# Autodesk Inventor assembly: 6 bar attachment_MIR
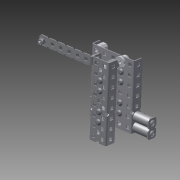
[picture p0: Inventor's stored thumbnail of the model, 180x180]
Saved by Autodesk Inventor 2014 SP1 (Build 180222100, 222)
## iProperties
Created: 2014-03-20
Part Number: 6 bar attachment_MIR
Document SubType Name: Assembly
Designer: Ryan
Author: Ryan
## Documents named in this file (16)
- C:\Users\Ryan\Desktop\sw\toss up 5th A bot\intake\6 bar attachment_MIR.iam
- C:\Users\Ryan\Desktop\sw\lib\Aperture VEX CAD Library\Metal\C Channel\5 x 7.ipt
- C:\Users\Ryan\Desktop\sw\lib\Aperture VEX CAD Library\Bearing Blocks\Bearing Block.ipt
- C:\Users\Ryan\Desktop\sw\lib\Aperture VEX CAD Library\Hardware\8-32\8-32_.500.ipt
- C:\Users\Ryan\Desktop\sw\lib\Aperture VEX CAD Library\Hardware\8-32\8-32 nylock.ipt
- C:\Users\Ryan\Desktop\sw\lib\Aperture VEX CAD Library\Metal\C Channel\2 x 8.ipt
- C:\Users\Ryan\Desktop\sw\lib\Aperture VEX CAD Library\Hardware\8-32\8-23_.750.ipt
- C:\Users\Ryan\Desktop\sw\lib\Aperture VEX CAD Library\Hardware\8-32\8-32 nylock_MIR14.ipt
- C:\Users\Ryan\Desktop\sw\lib\Aperture VEX CAD Library\Spacers\SPACER-0500-0375.ipt
- C:\Users\Ryan\Desktop\sw\lib\Aperture VEX CAD Library\Spacers\SPACER-0500-0250.ipt
- C:\Users\Ryan\Desktop\sw\lib\Aperture VEX CAD Library\Spacers\SPACER-0500-0125.ipt
- C:\Users\Ryan\Desktop\sw\lib\Aperture VEX CAD Library\Hardware\8-32\8-32_.375.ipt
- C:\Users\Ryan\Desktop\sw\lib\Aperture VEX CAD Library\Metal\Custom 1 bar\6 bend 1.ipt
- C:\Users\Ryan\Desktop\sw\lib\Aperture VEX CAD Library\Spacers\SPACER-0500-0500.ipt
- C:\Users\Ryan\Desktop\sw\lib\Aperture VEX CAD Library\Hardware\8-32\8-32_1.000.ipt
- C:\Users\Ryan\Desktop\sw\lib\Aperture VEX CAD Library\Metal\Custom 1 bar\1x2 bar.ipt
## Components (45 placed, 15 different names)
1. 5 x 7:1 — Mate:75, Mate:74, Mate:66, Mate:77, Mate:76, Mate:70, Mate:81, Mate:79, Mate:78, Mate:83, Flush:3, Flush:2, Mate:88, Mate:90, Mate:99, Mate:47, Mate:48, Mate:58, Mate:59, Mate:60, Mate:61, Flush:4
2. Bearing Block:1 — Mate:75, Mate:74, Mate:66, Mate:65, Mate:64, Mate:63, Mate:89
3. Bearing Block:2 — Mate:65, Mate:64, Mate:63, Mate:87, Mate:92, Mate:94, Mate:48
4. 2 x 8:1 — Flush:3, Flush:2, Mate:104, Mate:103, Mate:102, Flush:4, Mate:106
5. 8-23_.750:1 — Mate:88, Mate:87, Mate:91
6. 8-23_.750:2 — Mate:90, Mate:89, Mate:93
7. 8-32 nylock_MIR14:1 — Mate:92, Mate:91
8. 8-32 nylock:2 — Mate:94, Mate:93
9. SPACER-0500-0375:1 — Mate:96, Mate:95, Mate:101, Mate:49
10. SPACER-0500-0250:1 — Mate:96, Mate:95
11. SPACER-0500-0125:1 — Mate:101, Mate:100, Mate:99
12. 8-32_.375:1 — Mate:104, Mate:103, Mate:102, Mate:105, Mate:108, Mate:107
13. 8-32 nylock:3 — Mate:105, Mate:109
14. 6 bend 1:1 — Flush:4, Mate:109, Mate:108, Mate:107, Mate:106, Mate:112, Mate:111, Mate:110, Mate:114
15. 8-32_.375:2 — Mate:112, Mate:111, Mate:110, Mate:113
16. 8-32 nylock:4 — Mate:114, Mate:113
17. 1x2 bar:1 — Mate:56, Mate:57, Flush:4
18. Bearing Block:3 — Mate:77, Mate:76, Mate:70, Mate:82, Mate:85, Mate:100, Flush:3, Mate:47, Mate:49
19. Bearing Block:4 — Mate:81, Mate:79, Mate:78, Flush:3
20. Bearing Block:5
21. Bearing Block:6
22. 8-32_1.000:1 — Mate:56
23. SPACER-0500-0500:1 — Mate:57
24. SPACER-0500-0375:2 — Mate:59, Mate:60, Mate:61
25. 8-32 nylock:12 — Mate:58
26. 8-32_1.000:2
27. SPACER-0500-0500:2
28. SPACER-0500-0375:3
29. 8-32 nylock:13
30. 8-32_.500:1 — Mate:83, Mate:82, Mate:84
31. 8-32 nylock:1 — Mate:85, Mate:84
32. 8-32_.500:2
33. 8-32 nylock:5
34. 8-32_.500:3
35. 8-32 nylock:6
36. 8-32_.500:4
37. 8-32 nylock:7
38. 8-32_.500:5
39. 8-32 nylock:8
40. 8-32_.500:6
41. 8-32 nylock:9
42. 8-32_.500:7
43. 8-32 nylock:10
44. 8-32_.500:8
45. 8-32 nylock:11
## Component patterns: (2 elements, first: Bearing Block:3 + Bearing Block:4), (2 elements, first: 8-32_1.000:1 + SPACER-0500-0500:1 + SPACER-0500-0375:2 + 8-32 nylock:12), (4 elements, first: 8-32_.500:1 + 8-32 nylock:1), Component Pattern 1:2 (4 elements)
## Relationships (62: Mate 58, Flush 4)
- Mate:75 (2.3114 mm): 5 x 7:1 ↔ Bearing Block:1
- Mate:74 (2.3114 mm): 5 x 7:1 ↔ Bearing Block:1
- Mate:66: 5 x 7:1 ↔ Bearing Block:1
- Mate:65: Bearing Block:1 ↔ Bearing Block:2
- Mate:64: Bearing Block:1 ↔ Bearing Block:2
- Mate:63: Bearing Block:1 ↔ Bearing Block:2
- Mate:77 (2.3114 mm): 5 x 7:1 ↔ Bearing Block:3
- Mate:76 (2.3114 mm): 5 x 7:1 ↔ Bearing Block:3
- Mate:70: 5 x 7:1 ↔ Bearing Block:3
- Mate:81 (2.3114 mm): 5 x 7:1 ↔ Bearing Block:4
- Mate:79 (2.3114 mm): 5 x 7:1 ↔ Bearing Block:4
- Mate:78: 5 x 7:1 ↔ Bearing Block:4
- Mate:83: 5 x 7:1 ↔ 8-32_.500:1
- Mate:82: Bearing Block:3 ↔ 8-32_.500:1
- Mate:85: Bearing Block:3 ↔ 8-32 nylock:1
- Mate:84: 8-32_.500:1 ↔ 8-32 nylock:1
- Flush:3 [Mate]: 5 x 7:1 ↔ 2 x 8:1
- Flush:2: 5 x 7:1 ↔ 2 x 8:1
- Mate:88: 5 x 7:1 ↔ 8-23_.750:1
- Mate:87: Bearing Block:2 ↔ 8-23_.750:1
- Mate:90: 5 x 7:1 ↔ 8-23_.750:2
- Mate:89: Bearing Block:1 ↔ 8-23_.750:2
- Mate:92: Bearing Block:2 ↔ 8-32 nylock_MIR14:1
- Mate:91: 8-23_.750:1 ↔ 8-32 nylock_MIR14:1
- Mate:94: Bearing Block:2 ↔ 8-32 nylock:2
- Mate:93: 8-23_.750:2 ↔ 8-32 nylock:2
- Mate:96: SPACER-0500-0375:1 ↔ SPACER-0500-0250:1
- Mate:95: SPACER-0500-0375:1 ↔ SPACER-0500-0250:1
- Mate:101 (7.5184 mm): SPACER-0500-0375:1 ↔ SPACER-0500-0125:1
- Mate:100: SPACER-0500-0125:1 ↔ Bearing Block:3
- Mate:99: 5 x 7:1 ↔ SPACER-0500-0125:1
- Mate:104 (2.3114 mm): 2 x 8:1 ↔ 8-32_.375:1
- Mate:103: 2 x 8:1 ↔ 8-32_.375:1
- Mate:102 (2.3114 mm): 2 x 8:1 ↔ 8-32_.375:1
- Mate:105: 8-32_.375:1 ↔ 8-32 nylock:3
- Flush:4: 2 x 8:1 ↔ 6 bend 1:1
- Mate:109: 8-32 nylock:3 ↔ 6 bend 1:1
- Mate:108 (2.3114 mm): 8-32_.375:1 ↔ 6 bend 1:1
- Mate:107 (2.3114 mm): 8-32_.375:1 ↔ 6 bend 1:1
- Mate:106: 2 x 8:1 ↔ 6 bend 1:1
- Mate:112: 6 bend 1:1 ↔ 8-32_.375:2
- Mate:111 (2.3114 mm): 6 bend 1:1 ↔ 8-32_.375:2
- Mate:110 (2.3114 mm): 6 bend 1:1 ↔ 8-32_.375:2
- Mate:114 (1.1684 mm): 6 bend 1:1 ↔ 8-32 nylock:4
- Mate:113: 8-32_.375:2 ↔ 8-32 nylock:4
- Flush:3: Bearing Block:3 ↔ Bearing Block:4
- Mate:47 (2.3114 mm): 5 x 7:1 ↔ Bearing Block:3
- Mate:48 (2.3114 mm): 5 x 7:1 ↔ Bearing Block:2
- Mate:49: SPACER-0500-0375:1 ↔ Bearing Block:3
- [Mate]: SPACER-0500-0500:1 ↔ SPACER-0500-0375:2
- [Mate]: SPACER-0500-0500:1 ↔ SPACER-0500-0375:2
- [Mate]: 8-32_1.000:1 ↔ SPACER-0500-0500:1
- [Mate]: 1x2 bar:1 ↔ SPACER-0500-0500:1
- [Mate]: 1x2 bar:1 ↔ 8-32_1.000:1
- [Mate]: SPACER-0500-0375:2 ↔ 8-32 nylock:12
- Mate:56 (2.3114 mm): 1x2 bar:1 ↔ 8-32_1.000:1
- Mate:57 (2.3114 mm): 1x2 bar:1 ↔ SPACER-0500-0500:1
- Mate:58: 5 x 7:1 ↔ 8-32 nylock:12
- Mate:59: 5 x 7:1 ↔ SPACER-0500-0375:2
- Mate:60 (2.3114 mm): 5 x 7:1 ↔ SPACER-0500-0375:2
- Mate:61 (2.3114 mm): 5 x 7:1 ↔ SPACER-0500-0375:2
- Flush:4: 5 x 7:1 ↔ 1x2 bar:1
## Named parameters: q = 2.3114 mm
